(part 1 of 2)
# Autodesk Inventor assembly: #SHOOTER.3
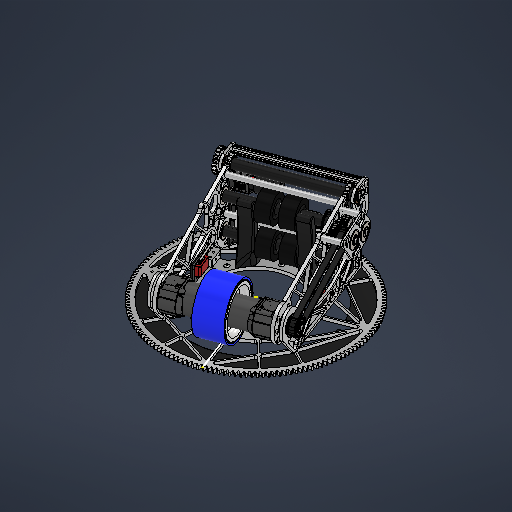
[picture p0: Inventor's stored thumbnail of the model, 512x512]
Saved by Autodesk Inventor 2026 (Build 300175000, 175)
## iProperties
Created: 2026-01-27
Part Number: #SHOOTER.3
Document SubType Name: Assembly
Designer: Owen L
Mass: 5085.84 g
Surface Area: 9899.41 cm^2
Volume: 1803.06 cm^3
Density: 2.82066 g/cm^3
Author: Owen L
## Documents named in this file (60)
- C:\Users\littl\OneDrive\Documents\GitHub\2026-Robot-Mechanical\Shooter\Shooter - Front Motors\#SHOOTER.FRONT_MOTORS.iam
- C:\Users\littl\OneDrive\Documents\GitHub\2026-Robot-Mechanical\Shooter\Shooter - Front Motors\PLATE,SHOOTER,SIDE.ipt
- C:\Users\littl\OneDrive\Documents\GitHub\2026-Robot-Mechanical\#1_CAD Library\Electronics\CONTROLS,SPARK_FLEX.ipt
- C:\Users\littl\OneDrive\Documents\GitHub\2026-Robot-Mechanical\#1_CAD Library\Power Transmission\Bushings\PURCHASED,BUSHING,13.75mmID,0.75inOD.ipt
- C:\Users\littl\OneDrive\Documents\GitHub\2026-Robot-Mechanical\#1_CAD Library\Power Transmission\Bearings\PURCHASED,HEX_BEARING.ipt
- C:\Users\littl\OneDrive\Documents\GitHub\2026-Robot-Mechanical\#1_CAD Library\Motors\MOTOR,REV,NEO,VORTEX.ipt
- C:\Users\littl\OneDrive\Documents\GitHub\2026-Robot-Mechanical\#1_CAD Library\Motors\MOTOR,REV,NEO,550.ipt
- C:\Users\littl\OneDrive\Documents\GitHub\2026-Robot-Mechanical\#1_CAD Library\Power Transmission\UltraPlanetary\PURCHASED,REV,ULTRAPLANETARY,2-STAGE.iam
- C:\Users\littl\OneDrive\Documents\GitHub\2026-Robot-Mechanical\Shooter\Shooter - Front Motors\#SHOOTER.3\Design Accelerator\PLATE,HOOD,SIDE.ipt
- C:\Users\littl\OneDrive\Documents\GitHub\2026-Robot-Mechanical\Shooter\Shooter - Front Motors\#SHOOTER.3\Design Accelerator\PLATE.HOOD,PINION,GEAR.ipt
- C:\Users\littl\OneDrive\Documents\GitHub\2026-Robot-Mechanical\Shooter\Shooter - Front Motors\STOCK,HEX,ROUND,HOOD.ipt
- C:\Users\littl\OneDrive\Documents\GitHub\2026-Robot-Mechanical\#1_CAD Library\Power Transmission\Pulleys\PURCHASED,HTD5mm,20T,PULLEY.ipt
- C:\Users\littl\OneDrive\Documents\GitHub\2026-Robot-Mechanical\Shooter\Shooter - Front Motors\#SHOOTER.3\Design Accelerator\PLATE,HOOD,DRIVE,GEAR,SHAFT.ipt
- C:\Users\littl\OneDrive\Documents\GitHub\2026-Robot-Mechanical\Shooter\Shooter - Front Motors\#SHOOTER.3\Design Accelerator\PLATE,HOOD,DRIVE,GEAR,MOTOR.ipt
- C:\Users\littl\OneDrive\Documents\GitHub\2026-Robot-Mechanical\Shooter\Shooter - Front Motors\STOCK,SHAFT,HEX,SHOOTER.ipt
- C:\Users\littl\OneDrive\Documents\GitHub\2026-Robot-Mechanical\Shooter\Shooter - Front Motors\PLATE,BEARING,MOUNT.ipt
- C:\Users\littl\OneDrive\Documents\GitHub\2026-Robot-Mechanical\Shooter\Shooter - Front Motors\STOCK,SHAFT,HEX,HOOD,WHEELS,LONG.ipt
- C:\Users\littl\OneDrive\Documents\GitHub\2026-Robot-Mechanical\Shooter\Shooter - Front Motors\STOCK,SHAFT,HEX,HOOD,REVERSER.ipt
- C:\Users\littl\OneDrive\Documents\GitHub\2026-Robot-Mechanical\Shooter\Shooter - Front Motors\STOCK,SHAFT,HEX,HOOD,WHEELS,SHORT.ipt
- C:\Users\littl\OneDrive\Documents\GitHub\2026-Robot-Mechanical\Shooter\Shooter - Front Motors\PLATE,SHOOTER,BOTTOM.ipt
- C:\Users\littl\OneDrive\Documents\GitHub\2026-Robot-Mechanical\Shooter\Shooter - Front Motors\PLATE,SHOOTER,BACK.ipt
- C:\Users\littl\OneDrive\Documents\GitHub\2026-Robot-Mechanical\Shooter\Shooter - Front Motors\STOCK,CHURRO,HEX,BACK.ipt
- C:\Users\littl\OneDrive\Documents\GitHub\2026-Robot-Mechanical\Shooter\Shooter - Front Motors\PURCHASED,WASHER.ipt
- C:\Users\littl\OneDrive\Documents\GitHub\2026-Robot-Mechanical\#1_CAD Library\Wheels\Shooter\PURCHASED,2inOD,HEX,SHOOTER,WHEEL.ipt
- C:\Users\littl\OneDrive\Documents\GitHub\2026-Robot-Mechanical\#1_CAD Library\Building Materials\Fasteners\Bolts\PURCHASED,0.25-20x0.5in,BUTTONHEAD,BOLT.ipt
- C:\Users\littl\OneDrive\Documents\GitHub\2026-Robot-Mechanical\#1_CAD Library\Building Materials\Fasteners\Bolts\PURCHASED,10-32x0.5in,BUTTONHEAD,BOLT.ipt
- C:\Users\littl\OneDrive\Documents\GitHub\2026-Robot-Mechanical\#1_CAD Library\Building Materials\Fasteners\Bolts\PURCHASED,M3x10mm,BUTTONHEAD,BOLT.ipt
- C:\Users\littl\OneDrive\Documents\GitHub\2026-Robot-Mechanical\Shooter\Shooter - Front Motors\3DPRINT,HOOD,DRIVEGEAR,SPACER.ipt
- C:\Users\littl\OneDrive\Documents\GitHub\2026-Robot-Mechanical\Shooter\Shooter - Front Motors\3DPRINT,REVERSERGEAR,SPACER.ipt
- C:\Users\littl\OneDrive\Documents\GitHub\2026-Robot-Mechanical\Shooter\Shooter - Front Motors\3DPRINT,BACKROLLERS,OPENSIDE,SPACER.ipt
- C:\Users\littl\OneDrive\Documents\GitHub\2026-Robot-Mechanical\Shooter\Shooter - Front Motors\3DPRINT,BACKROLLERS,PULLEYSIDE,SPACER.ipt
- C:\Users\littl\OneDrive\Documents\GitHub\2026-Robot-Mechanical\Shooter\Shooter - Front Motors\3DPRINT,BACKROLLERS,INTERROLLER,SPACER.ipt
- C:\Users\littl\OneDrive\Documents\GitHub\2026-Robot-Mechanical\#1_CAD Library\Power Transmission\Gears\PURCHASED,GEAR,20DP,30T,HEX.ipt
- C:\Users\littl\OneDrive\Documents\GitHub\2026-Robot-Mechanical\Shooter\Shooter - Front Motors\3DPRINT,BACKRAIL.ipt
- C:\Users\littl\OneDrive\Documents\GitHub\2026-Robot-Mechanical\Shooter\Shooter - Front Motors\3DPRINT,BACKRAIL_MIR.ipt
- C:\Users\littl\OneDrive\Documents\GitHub\2026-Robot-Mechanical\Shooter\Shooter - Front Motors\PLATE,NUTBLOCK.ipt
- C:\Users\littl\OneDrive\Documents\GitHub\2026-Robot-Mechanical\#1_CAD Library\Building Materials\Fasteners\Bolts\PURCHASED,M4x12mm,BUTTONHEAD,BOLT.ipt
- C:\Users\littl\OneDrive\Documents\GitHub\2026-Robot-Mechanical\Shooter\Shooter - Front Motors\STANDIN,45T,HTD5mm,BELT.ipt
- C:\Users\littl\OneDrive\Documents\GitHub\2026-Robot-Mechanical\Shooter\Shooter - Front Motors\STANDIN,90T,HTD5mm,BELT.ipt
- C:\Users\littl\OneDrive\Documents\GitHub\2026-Robot-Mechanical\Shooter\Shooter - Front Motors\3DPRINT,FLYWHEELTOHOOD,SPACER.ipt
- C:\Users\littl\OneDrive\Documents\GitHub\2026-Robot-Mechanical\Shooter\Shooter - Front Motors\STOCK,HOOD,SPACER,10-32,6.25in.ipt
- C:\Users\littl\OneDrive\Documents\GitHub\2026-Robot-Mechanical\Shooter\Shooter - Front Motors\3DPRINT,SIDEPLATETOHOOD,SPACER .ipt
- C:\Users\littl\OneDrive\Documents\GitHub\2026-Robot-Mechanical\Shooter\Shooter - Front Motors\3DPRINT,SIDEPLATETOHOODGEAR,SPACER.ipt
- C:\Users\littl\OneDrive\Documents\GitHub\2026-Robot-Mechanical\Shooter\Shooter - Front Motors\3DPRINT,BUSHINGTOHOODDRIVEGEAR,SPACER.ipt
- C:\Users\littl\OneDrive\Documents\GitHub\2026-Robot-Mechanical\Shooter\Shooter - Front Motors\3DPRINT,HOOD,ALIGNMENT,PLATES.ipt
- C:\Users\littl\OneDrive\Documents\GitHub\2026-Robot-Mechanical\#1_CAD Library\Building Materials\Fasteners\Bolts\PURCHASED,M3x16mm,BUTTONHEAD,BOLT.ipt
- C:\Users\littl\OneDrive\Documents\GitHub\2026-Robot-Mechanical\#1_CAD Library\Building Materials\Fasteners\Nuts\PURCHASED,M3,NYLOCK,NUT.ipt
- C:\Users\littl\OneDrive\Documents\GitHub\2026-Robot-Mechanical\#1_CAD Library\Electronics\CONTROLS,LIMIT_SWITCH,VEX.iam
- C:\Users\littl\OneDrive\Documents\GitHub\2026-Robot-Mechanical\Shooter\Shooter - Front Motors\3DPRINT,LIMIT_SWITCH,SPACER.ipt
- C:\Users\littl\OneDrive\Documents\GitHub\2026-Robot-Mechanical\Shooter\Shooter - Front Motors\3DPRINT,LIMIT_SWITCH,SPACER,RIGHT.ipt
- C:\Users\littl\OneDrive\Documents\GitHub\2026-Robot-Mechanical\Shooter\Shooter - Front Motors\PLATE,FLYWHEEL,HUB.ipt
- C:\Users\littl\OneDrive\Documents\GitHub\2026-Robot-Mechanical\Shooter\Shooter - Front Motors\CAST,FLYWHEEL,GRIP.ipt
- C:\Users\littl\OneDrive\Documents\GitHub\2026-Robot-Mechanical\#1_CAD Library\Electronics\CONTROLS,SPARK_MAX.ipt
- C:\Users\littl\OneDrive\Documents\GitHub\2026-Robot-Mechanical\Shooter\Shooter - Front Motors\3DPRINT,SPARK_MAX,MOUNT.ipt
- C:\Users\littl\OneDrive\Documents\GitHub\2026-Robot-Mechanical\#1_CAD Library\Building Materials\Fasteners\Bolts\PURCHASED,10-32x0.625in,FLATHEAD,BOLT.ipt
- C:\Users\littl\OneDrive\Documents\GitHub\2026-Robot-Mechanical\Shooter\Shooter - Front Motors\3DPRINT,REVERSERGEAR,SPACER,SHORT.ipt
- C:\Users\littl\OneDrive\Documents\GitHub\2026-Robot-Mechanical\Shooter\Shooter - Front Motors\3DPRINT,CABLE,GUARD.ipt
- C:\Users\littl\OneDrive\Documents\GitHub\2026-Robot-Mechanical\Shooter\Shooter - Front Motors\3DPRINT,BACKROLLERS,PULLEY,SPACER.ipt
- C:\Users\littl\OneDrive\Documents\GitHub\2026-Robot-Mechanical\Shooter\Shooter - Front Motors\PLATE,NUTBLOCK,BACK.ipt
- C:\Users\littl\OneDrive\Documents\GitHub\2026-Robot-Mechanical\Shooter\Shooter - Front Motors\STOCK,ROUND,0.375inOD,10-32,STANDOFF.ipt
## Components (209 placed, 59 different names)
1. STOCK,ROUND,0.375inOD,10-32,STANDOFF:1 — Insert:243
2. STOCK,ROUND,0.375inOD,10-32,STANDOFF:2 — Insert:244
3. STOCK,ROUND,0.375inOD,10-32,STANDOFF:3 — Insert:245
4. PLATE,NUTBLOCK,BACK:1 — Insert:238, Insert:239
5. PLATE,NUTBLOCK:1 — Insert:101, Insert:102
6. PLATE,NUTBLOCK:2 — Insert:103, Insert:104
7. PLATE,NUTBLOCK:4 — Insert:107, Mate:181
8. PLATE,NUTBLOCK:5 — Insert:110, Mate:193
9. STANDIN,45T,HTD5mm,BELT:1 — Mate:147, Mate:148, Mate:152
10. STANDIN,90T,HTD5mm,BELT:1 — Mate:149, Mate:150, Mate:151
11. CONTROLS,SPARK_FLEX:1 — Mate:3, Mate:4, Mate:5, Insert:188, Insert:219
12. CONTROLS,SPARK_FLEX:2 — Mate:12, Mate:13, Mate:14, Insert:191, Insert:220
13. MOTOR,REV,NEO,VORTEX:1 — Mate:3, Mate:4, Mate:5
14. MOTOR,REV,NEO,VORTEX:2 — Mate:12, Mate:13, Mate:14, Mate:209
15. MOTOR,REV,NEO,550:1 — Insert:1, Mate:1
16. CONTROLS,SPARK_MAX:1 — Mate:216, Mate:220, Mate:221
17. CONTROLS,LIMIT_SWITCH,VEX:2 [sub-assembly] — Mate:198, Mate:199, Mate:200, Mate:203, Mate:204
18. CONTROLS,LIMIT_SWITCH,VEX:1 [sub-assembly] — Mate:184, Mate:185, Mate:186, Mate:188, Mate:190
19. PURCHASED,BUSHING,13.75mmID,0.75inOD:1 — Insert:3, Mate:8, Mate:166, Mate:173
20. PURCHASED,BUSHING,13.75mmID,0.75inOD:2 — Insert:7, Mate:11, Mate:170
21. PURCHASED,HEX_BEARING:1 — Insert:4, Mate:30, Mate:31, Mate:191, Mate:192
22. PURCHASED,REV,ULTRAPLANETARY,2-STAGE:1 [sub-assembly] — Insert:1, Mate:1, Insert:2, Mate:2, Flush:1, Insert:14, Mate:26
23. PURCHASED,HTD5mm,20T,PULLEY:1 — Mate:59, Mate:60, Mate:97, Mate:152, Mate:248
24. PURCHASED,HEX_BEARING:5 — Insert:15, Mate:37, Mate:38, Flush:3, Mate:194
25. PURCHASED,HEX_BEARING:6 — Insert:16, Mate:39, Mate:40, Flush:4
26. PURCHASED,HEX_BEARING:7 — Insert:17, Mate:128
27. PURCHASED,HEX_BEARING:8 — Insert:18
28. PURCHASED,HEX_BEARING:9 — Insert:19, Mate:155
29. PURCHASED,HEX_BEARING:10 — Insert:20, Mate:162
30. PURCHASED,HEX_BEARING:11 — Insert:21, Mate:159
31. PURCHASED,HEX_BEARING:12 — Mate:41, Mate:42, Flush:5, Mate:129, Insert:231
32. PURCHASED,HEX_BEARING:14 — Mate:88, Mate:121, Mate:122, Insert:96
33. PURCHASED,HEX_BEARING:15 — Insert:94, Mate:226
34. PURCHASED,HTD5mm,20T,PULLEY:2 — Mate:61, Mate:62, Mate:100, Mate:246
35. PURCHASED,2inOD,HEX,SHOOTER,WHEEL:1 — Mate:65, Mate:66, Mate:73, Mate:103, Mate:243
36. PURCHASED,2inOD,HEX,SHOOTER,WHEEL:2 — Mate:67, Mate:68, Mate:73, Flush:8, Mate:91
37. PURCHASED,2inOD,HEX,SHOOTER,WHEEL:3 — Mate:69, Mate:70, Mate:74, Mate:106, Mate:244
38. PURCHASED,2inOD,HEX,SHOOTER,WHEEL:4 — Mate:71, Mate:72, Mate:74, Flush:8, Mate:94
39. PURCHASED,WASHER:12 — Insert:86, Insert:87
40. PURCHASED,GEAR,20DP,30T,HEX:1 — Mate:124, Mate:125, Mate:129, Mate:146
41. PURCHASED,GEAR,20DP,30T,HEX:2 — Mate:126, Mate:127, Mate:128
42. PURCHASED,HTD5mm,20T,PULLEY:3 — Mate:141, Mate:142, Flush:9
43. PURCHASED,HTD5mm,20T,PULLEY:4 — Mate:144, Mate:145, Mate:146, Mate:151, Mate:227
44. 3DPRINT,BACKROLLERS,PULLEY,SPACER:1 — Mate:245, Mate:246, Mate:250
45. 3DPRINT,BACKROLLERS,PULLEY,SPACER:2 — Mate:247, Mate:248, Mate:249
46. 3DPRINT,CABLE,GUARD:1 — Mate:228, Mate:229, Mate:230, Mate:237, Mate:238
47. 3DPRINT,CABLE,GUARD:2 — Mate:228, Mate:229, Mate:230, Mate:231, Mate:232, Mate:233
48. 3DPRINT,CABLE,GUARD:3 — Mate:231, Mate:232, Mate:233, Mate:234, Mate:235, Mate:236
49. 3DPRINT,CABLE,GUARD:4 — Mate:234, Mate:235, Mate:236, Mate:239
50. 3DPRINT,HOOD,DRIVEGEAR,SPACER:1 — Mate:83, Mate:84, Mate:85, Mate:163
51. 3DPRINT,REVERSERGEAR,SPACER:1 — Mate:86, Mate:87, Mate:88
52. 3DPRINT,BACKROLLERS,OPENSIDE,SPACER:1 — Mate:89, Mate:90, Mate:91, Mate:194
53. 3DPRINT,BACKROLLERS,OPENSIDE,SPACER:2 — Mate:92, Mate:93, Mate:94
54. 3DPRINT,BACKROLLERS,PULLEYSIDE,SPACER:1 — Mate:95, Mate:96, Mate:97, Mate:243
55. 3DPRINT,BACKROLLERS,PULLEYSIDE,SPACER:2 — Mate:98, Mate:99, Mate:100, Mate:244
56. 3DPRINT,BACKROLLERS,INTERROLLER,SPACER:1 — Mate:101, Mate:102, Mate:103
57. 3DPRINT,BACKROLLERS,INTERROLLER,SPACER:2 — Mate:104, Mate:105, Mate:106
58. 3DPRINT,BACKRAIL:1 — Mate:131, Mate:212, Mate:225
59. 3DPRINT,BACKRAIL_MIR:1 — Mate:240, Mate:241, Mate:242
60. 3DPRINT,FLYWHEELTOHOOD,SPACER:1 — Mate:153, Mate:154, Mate:155
61. 3DPRINT,SIDEPLATETOHOOD,SPACER :1 — Mate:157, Mate:158, Mate:159
62. 3DPRINT,SIDEPLATETOHOODGEAR,SPACER:1 — Mate:171, Mate:172, Mate:173
63. 3DPRINT,BUSHINGTOHOODDRIVEGEAR,SPACER:1 — Mate:164, Mate:165, Mate:166, Mate:167
64. 3DPRINT,SIDEPLATETOHOOD,SPACER :2 — Mate:160, Mate:161, Mate:162, Mate:192
65. 3DPRINT,BUSHINGTOHOODDRIVEGEAR,SPACER:2 — Mate:168, Mate:169, Mate:170
66. 3DPRINT,HOOD,ALIGNMENT,PLATES:1 — Insert:161, Insert:165, Insert:174, Insert:175, Insert:176, Insert:177, Insert:178
67. 3DPRINT,HOOD,ALIGNMENT,PLATES:2 — Insert:163, Insert:164, Insert:179, Insert:180, Insert:181, Insert:182, Insert:183
68. 3DPRINT,HOOD,ALIGNMENT,PLATES:3 — Insert:166, Insert:167, Insert:170, Insert:171, Insert:172, Insert:173
69. 3DPRINT,HOOD,ALIGNMENT,PLATES:4 — Insert:168, Insert:169, Insert:184, Insert:185, Insert:186, Insert:187
70. 3DPRINT,LIMIT_SWITCH,SPACER:1 — Mate:181, Mate:182, Mate:183, Mate:184, Mate:186, Flush:10
71. 3DPRINT,LIMIT_SWITCH,SPACER,RIGHT:1 — Mate:196, Mate:197, Mate:198, Mate:199, Mate:200, Flush:10
72. 3DPRINT,SPARK_MAX,MOUNT:1 — Mate:217, Mate:218, Mate:220, Mate:221, Mate:224, Insert:240, Insert:241, Insert:242
73. 3DPRINT,REVERSERGEAR,SPACER,SHORT:1 — Mate:226, Mate:227
74. PURCHASED,10-32x0.5in,BUTTONHEAD,BOLT:78 — Insert:240
75. PURCHASED,10-32x0.5in,BUTTONHEAD,BOLT:79 — Insert:241
76. PURCHASED,10-32x0.5in,BUTTONHEAD,BOLT:80 — Insert:242
77. PURCHASED,WASHER:2 — Insert:47, Insert:62
78. PURCHASED,WASHER:3 — Insert:48, Insert:64
79. PURCHASED,WASHER:4 — Insert:49, Insert:63
80. PURCHASED,WASHER:5 — Insert:50, Insert:65, Mate:191
81. PURCHASED,WASHER:6 — Insert:51, Insert:66
82. PURCHASED,WASHER:7 — Insert:52, Insert:67
83. PURCHASED,WASHER:8 — Insert:53, Insert:68
84. PURCHASED,WASHER:9 — Insert:54, Insert:69
85. PURCHASED,WASHER:10 — Insert:55, Insert:70
86. PURCHASED,M3,NYLOCK,NUT:3 — Insert:187
87. PURCHASED,M3,NYLOCK,NUT:5 — Insert:185
88. PURCHASED,M3,NYLOCK,NUT:6 — Insert:184
89. PURCHASED,M3,NYLOCK,NUT:7 — Insert:183
90. PURCHASED,M3,NYLOCK,NUT:1 — Insert:186
91. PURCHASED,M3,NYLOCK,NUT:8 — Insert:182
92. PURCHASED,M3,NYLOCK,NUT:9 — Insert:181
93. PURCHASED,M3,NYLOCK,NUT:10 — Insert:180
94. PURCHASED,M3,NYLOCK,NUT:11 — Insert:179
95. PURCHASED,0.25-20x0.5in,BUTTONHEAD,BOLT:1 — Insert:146
96. PURCHASED,0.25-20x0.5in,BUTTONHEAD,BOLT:4 — Insert:145
97. PURCHASED,M3x10mm,BUTTONHEAD,BOLT:1 — Insert:77
98. PURCHASED,10-32x0.5in,BUTTONHEAD,BOLT:6 — Insert:62
99. PURCHASED,10-32x0.5in,BUTTONHEAD,BOLT:7 — Insert:63
100. PURCHASED,10-32x0.5in,BUTTONHEAD,BOLT:8 — Insert:65
101. PURCHASED,10-32x0.5in,BUTTONHEAD,BOLT:9 — Insert:64
102. PURCHASED,10-32x0.5in,BUTTONHEAD,BOLT:10 — Insert:66
103. PURCHASED,10-32x0.5in,BUTTONHEAD,BOLT:11 — Insert:67
104. PURCHASED,10-32x0.5in,BUTTONHEAD,BOLT:12 — Insert:68
105. PURCHASED,10-32x0.5in,BUTTONHEAD,BOLT:13 — Insert:69
106. PURCHASED,10-32x0.5in,BUTTONHEAD,BOLT:14 — Insert:70
107. PURCHASED,10-32x0.5in,BUTTONHEAD,BOLT:16 — Insert:87
108. PURCHASED,M3x10mm,BUTTONHEAD,BOLT:2 — Insert:78
109. PURCHASED,M3x10mm,BUTTONHEAD,BOLT:3 — Insert:80
110. PURCHASED,M3x10mm,BUTTONHEAD,BOLT:4 — Insert:79
111. PURCHASED,M3x10mm,BUTTONHEAD,BOLT:5 — Insert:81
112. PURCHASED,M3x10mm,BUTTONHEAD,BOLT:6 — Insert:82
113. PURCHASED,M3x10mm,BUTTONHEAD,BOLT:7 — Insert:83
114. PURCHASED,M3x10mm,BUTTONHEAD,BOLT:8 — Insert:84
115. PURCHASED,M3x10mm,BUTTONHEAD,BOLT:9 — Insert:85
116. PURCHASED,10-32x0.5in,BUTTONHEAD,BOLT:21 — Insert:99
117. PURCHASED,10-32x0.5in,BUTTONHEAD,BOLT:22 — Insert:98
118. PURCHASED,10-32x0.5in,BUTTONHEAD,BOLT:23 — Insert:100
119. PURCHASED,10-32x0.5in,BUTTONHEAD,BOLT:24 — Insert:91
120. PURCHASED,10-32x0.5in,BUTTONHEAD,BOLT:25 — Insert:92
121. PURCHASED,10-32x0.5in,BUTTONHEAD,BOLT:26 — Insert:93
122. PURCHASED,10-32x0.5in,BUTTONHEAD,BOLT:27 — Insert:114
123. PURCHASED,10-32x0.5in,BUTTONHEAD,BOLT:28 — Insert:113
124. PURCHASED,10-32x0.5in,BUTTONHEAD,BOLT:29 — Insert:112
125. PURCHASED,10-32x0.5in,BUTTONHEAD,BOLT:30 — Insert:111
126. PURCHASED,10-32x0.5in,BUTTONHEAD,BOLT:31 — Insert:115
127. PURCHASED,10-32x0.5in,BUTTONHEAD,BOLT:32 — Insert:116
128. PURCHASED,10-32x0.5in,BUTTONHEAD,BOLT:33 — Insert:117
129. PURCHASED,10-32x0.5in,BUTTONHEAD,BOLT:34 — Insert:118
130. PURCHASED,10-32x0.5in,BUTTONHEAD,BOLT:35 — Insert:119
131. PURCHASED,10-32x0.5in,BUTTONHEAD,BOLT:36 — Insert:120
132. PURCHASED,10-32x0.5in,BUTTONHEAD,BOLT:37 — Insert:121
133. PURCHASED,10-32x0.5in,BUTTONHEAD,BOLT:38 — Insert:122
134. PURCHASED,10-32x0.5in,BUTTONHEAD,BOLT:40 — Insert:124
135. PURCHASED,10-32x0.5in,BUTTONHEAD,BOLT:41 — Insert:125
136. PURCHASED,10-32x0.5in,BUTTONHEAD,BOLT:42 — Insert:126
137. PURCHASED,10-32x0.5in,BUTTONHEAD,BOLT:43 — Insert:127
138. PURCHASED,10-32x0.5in,BUTTONHEAD,BOLT:44 — Insert:128
139. PURCHASED,10-32x0.5in,BUTTONHEAD,BOLT:45 — Insert:129
140. PURCHASED,M4x12mm,BUTTONHEAD,BOLT:1 — Insert:137, Insert:232
141. PURCHASED,M4x12mm,BUTTONHEAD,BOLT:2 — Insert:138, Mate:212
142. PURCHASED,M4x12mm,BUTTONHEAD,BOLT:3 — Insert:139, Insert:234
143. PURCHASED,M4x12mm,BUTTONHEAD,BOLT:4 — Insert:140, Insert:233
144. PURCHASED,M4x12mm,BUTTONHEAD,BOLT:5 — Insert:141, Insert:237
145. PURCHASED,M4x12mm,BUTTONHEAD,BOLT:6 — Insert:142
146. PURCHASED,M4x12mm,BUTTONHEAD,BOLT:7 — Insert:143, Insert:236
147. PURCHASED,M4x12mm,BUTTONHEAD,BOLT:8 — Insert:144, Insert:235
148. PURCHASED,10-32x0.5in,BUTTONHEAD,BOLT:49 — Insert:154
149. PURCHASED,10-32x0.5in,BUTTONHEAD,BOLT:50 — Insert:156
150. PURCHASED,10-32x0.5in,BUTTONHEAD,BOLT:51 — Insert:155
151. PURCHASED,10-32x0.5in,BUTTONHEAD,BOLT:52 — Insert:157
152. PURCHASED,M3x16mm,BUTTONHEAD,BOLT:1 — Insert:170
153. PURCHASED,M3x16mm,BUTTONHEAD,BOLT:2 — Insert:171
154. PURCHASED,M3x16mm,BUTTONHEAD,BOLT:3 — Insert:172
155. PURCHASED,M3x16mm,BUTTONHEAD,BOLT:4 — Insert:173
156. PURCHASED,M3x16mm,BUTTONHEAD,BOLT:5 — Insert:174
157. PURCHASED,M3x16mm,BUTTONHEAD,BOLT:6 — Insert:175
158. PURCHASED,M3x16mm,BUTTONHEAD,BOLT:7 — Insert:176
159. PURCHASED,M3x16mm,BUTTONHEAD,BOLT:8 — Insert:177
160. PURCHASED,M3x16mm,BUTTONHEAD,BOLT:9 — Insert:178
161. PURCHASED,M4x12mm,BUTTONHEAD,BOLT:9 — Mate:187, Mate:188
162. PURCHASED,M4x12mm,BUTTONHEAD,BOLT:10 — Mate:189, Mate:190
163. PURCHASED,10-32x0.5in,BUTTONHEAD,BOLT:53 — Insert:195
164. PURCHASED,10-32x0.5in,BUTTONHEAD,BOLT:56 — Insert:198
165. PURCHASED,10-32x0.5in,BUTTONHEAD,BOLT:57 — Insert:201
166. PURCHASED,10-32x0.5in,BUTTONHEAD,BOLT:58 — Insert:200
167. PURCHASED,10-32x0.5in,BUTTONHEAD,BOLT:59 — Insert:199
168. PURCHASED,10-32x0.5in,BUTTONHEAD,BOLT:60 — Insert:203
169. PURCHASED,10-32x0.5in,BUTTONHEAD,BOLT:61 — Insert:204
170. PURCHASED,10-32x0.5in,BUTTONHEAD,BOLT:62 — Insert:202
171. PURCHASED,10-32x0.5in,BUTTONHEAD,BOLT:63 — Insert:205
172. PURCHASED,10-32x0.5in,BUTTONHEAD,BOLT:64 — Insert:207
173. PURCHASED,10-32x0.5in,BUTTONHEAD,BOLT:65 — Insert:208
174. PURCHASED,10-32x0.5in,BUTTONHEAD,BOLT:66 — Insert:206
175. PURCHASED,10-32x0.5in,BUTTONHEAD,BOLT:67 — Insert:210
176. PURCHASED,10-32x0.5in,BUTTONHEAD,BOLT:68 — Insert:209
177. PURCHASED,M4x12mm,BUTTONHEAD,BOLT:11 — Mate:201, Mate:204
178. PURCHASED,M4x12mm,BUTTONHEAD,BOLT:12 — Mate:202, Mate:203
179. PURCHASED,10-32x0.625in,FLATHEAD,BOLT:1 — Insert:221
180. PURCHASED,10-32x0.5in,BUTTONHEAD,BOLT:69 — Insert:222
181. PURCHASED,10-32x0.5in,BUTTONHEAD,BOLT:70 — Insert:223
182. PURCHASED,10-32x0.5in,BUTTONHEAD,BOLT:71 — Insert:224
183. PURCHASED,10-32x0.5in,BUTTONHEAD,BOLT:72 — Insert:225
184. PURCHASED,10-32x0.5in,BUTTONHEAD,BOLT:73 — Insert:226
185. PURCHASED,10-32x0.5in,BUTTONHEAD,BOLT:74 — Insert:227
186. PURCHASED,10-32x0.5in,BUTTONHEAD,BOLT:75 — Insert:228
187. PURCHASED,10-32x0.5in,BUTTONHEAD,BOLT:76 — Insert:229
188. PURCHASED,10-32x0.5in,BUTTONHEAD,BOLT:77 — Insert:230
189. PLATE,FLYWHEEL,HUB:1 — Mate:207, Mate:208, Mate:209, Mate:214, Flush:12, Mate:215
190. PLATE,HOOD,SIDE:1 — Mate:6, Mate:7, Mate:15, Insert:15, Insert:16, Mate:27, Insert:20, Insert:152, Insert:154, Insert:155, Mate:174, Insert:161, Insert:163, Insert:164, Insert:165, Insert:188, Insert:205, Insert:206, Insert:207, Insert:208, Insert:209, Insert:210, Insert:219
191. PLATE.HOOD,PINION,GEAR:1 — Mate:22, Mate:23, Mate:163, Mate:167
192. PLATE,HOOD,SIDE:2 — Mate:7, Mate:15, Insert:17, Insert:18, Mate:27, Insert:21, Insert:91, Insert:92, Insert:93, Mate:147, Mate:148, Mate:150, Insert:153, Insert:156, Insert:157, Insert:166, Insert:167, Insert:168, Insert:169, Insert:191, Insert:199, Insert:200, Insert:201, Insert:202, Insert:203, Insert:204, Insert:220, Insert:231, Insert:243, Insert:244, Insert:245
193. PLATE.HOOD,PINION,GEAR:2 — Mate:20, Mate:21, Mate:85
194. PLATE,HOOD,DRIVE,GEAR,SHAFT:1 — Mate:24, Mate:25, Flush:2
195. PLATE,HOOD,DRIVE,GEAR,MOTOR:1 — Insert:14, Mate:26, Flush:2, Insert:77, Insert:78, Insert:79, Insert:80, Insert:81
196. PLATE,SHOOTER,SIDE:1 — Insert:2, Mate:2, Insert:3, Insert:4, Mate:6, Mate:36, Insert:82, Insert:83, Insert:84, Insert:85, Mate:120, Insert:110, Insert:111, Insert:112, Insert:113, Insert:114, Insert:146, Mate:182, Mate:187, Mate:189, Insert:195, Insert:229
197. PLATE,SHOOTER,BACK:1 — Insert:128, Insert:129, Insert:192, Insert:193, Mate:216, Mate:217, Mate:218, Mate:224, Insert:238, Insert:239
198. PLATE,SHOOTER,BOTTOM:1 — Mate:120, Mate:131, Insert:102, Insert:103, Insert:107, Insert:115, Insert:116, Insert:117, Insert:118, Insert:119, Insert:120, Insert:121, Insert:122, Insert:137, Insert:138, Insert:139, Insert:140, Insert:141, Insert:142, Insert:143, Insert:144, Mate:174, Mate:183, Mate:185, Mate:193, Mate:210, Mate:211, Mate:225, Insert:221, Insert:222, Insert:223, Insert:224, Insert:225, Insert:226, Insert:227, Insert:228, Mate:237, Mate:238, Mate:239, Insert:232, Insert:233, Insert:234, Insert:235, Insert:236, Insert:237, Mate:240, Mate:241, Mate:242
199. PLATE,BEARING,MOUNT:1 — Insert:94, Insert:96, Insert:98, Insert:99, Insert:100
200. PLATE,SHOOTER,SIDE:2 — Insert:7, Insert:19, Mate:36, Insert:40, Insert:101, Insert:104, Insert:124, Insert:125, Insert:126, Insert:127, Insert:145, Mate:149, Insert:192, Insert:193, Insert:198, Mate:196, Mate:197, Mate:201, Mate:202, Insert:230
201. STOCK,HEX,ROUND,HOOD:1 — Mate:8, Flush:1, Mate:11, Mate:20, Mate:21, Mate:22, Mate:23, Mate:24, Mate:25, Insert:47, Insert:55, Mate:83, Mate:84, Mate:164, Mate:165, Mate:168, Mate:169, Mate:171, Mate:172
202. STOCK,SHAFT,HEX,SHOOTER:1 — Mate:30, Mate:31, Insert:50, Insert:51, Mate:141, Mate:142, Flush:9, Mate:153, Mate:154, Mate:157, Mate:158, Mate:160, Mate:161, Mate:207, Mate:208, Rotation:4
203. STOCK,SHAFT,HEX,HOOD,WHEELS,LONG:1 — Mate:37, Mate:38, Flush:3, Mate:59, Mate:60, Insert:48, Insert:53, Mate:65, Mate:66, Mate:67, Mate:68, Mate:86, Mate:87, Mate:89, Mate:90, Mate:95, Mate:96, Mate:101, Mate:102, Mate:121, Mate:122, Mate:126, Mate:127, Rotation:1, Rotation:2, Rotation:3, Mate:247, Mate:249
204. STOCK,SHAFT,HEX,HOOD,REVERSER:1 — Mate:41, Mate:42, Flush:5, Insert:52, Insert:86, Mate:124, Mate:125, Mate:144, Mate:145, Rotation:1, Rotation:2, Rotation:4
205. STOCK,SHAFT,HEX,HOOD,WHEELS,SHORT:1 — Mate:39, Mate:40, Flush:4, Mate:61, Mate:62, Insert:49, Insert:54, Mate:69, Mate:70, Mate:71, Mate:72, Mate:92, Mate:93, Mate:98, Mate:99, Mate:104, Mate:105, Rotation:3, Mate:245, Mate:250
206. STOCK,CHURRO,HEX,BACK:1 — Insert:40
207. STOCK,HOOD,SPACER,10-32,6.25in:1 — Insert:152
208. STOCK,HOOD,SPACER,10-32,6.25in:2 — Insert:153
209. CAST,FLYWHEEL,GRIP:2 — Mate:214, Flush:12, Mate:215
## Relationships (348: Mate 173, Insert 162, Flush 9, RelateRotation 4)
- Insert:1: MOTOR,REV,NEO,550:1 ↔ PURCHASED,REV,ULTRAPLANETARY,2-STAGE:1
- Mate:1: MOTOR,REV,NEO,550:1 ↔ PURCHASED,REV,ULTRAPLANETARY,2-STAGE:1
- Insert:2: PURCHASED,REV,ULTRAPLANETARY,2-STAGE:1 ↔ PLATE,SHOOTER,SIDE:1
- Mate:2: PURCHASED,REV,ULTRAPLANETARY,2-STAGE:1 ↔ PLATE,SHOOTER,SIDE:1
- Insert:3: PURCHASED,BUSHING,13.75mmID,0.75inOD:1 ↔ PLATE,SHOOTER,SIDE:1
- Insert:4: PURCHASED,HEX_BEARING:1 ↔ PLATE,SHOOTER,SIDE:1
- Mate:3: CONTROLS,SPARK_FLEX:1 ↔ MOTOR,REV,NEO,VORTEX:1
- Mate:4: CONTROLS,SPARK_FLEX:1 ↔ MOTOR,REV,NEO,VORTEX:1
- Mate:5: CONTROLS,SPARK_FLEX:1 ↔ MOTOR,REV,NEO,VORTEX:1
- Mate:6: PLATE,HOOD,SIDE:1 ↔ PLATE,SHOOTER,SIDE:1
- Mate:7 (177.8 mm): PLATE,HOOD,SIDE:1 ↔ PLATE,HOOD,SIDE:2
- Mate:8: PURCHASED,BUSHING,13.75mmID,0.75inOD:1 ↔ STOCK,HEX,ROUND,HOOD:1
- Flush:1 (-6.35 mm): PURCHASED,REV,ULTRAPLANETARY,2-STAGE:1 ↔ STOCK,HEX,ROUND,HOOD:1
- Insert:7: PURCHASED,BUSHING,13.75mmID,0.75inOD:2 ↔ PLATE,SHOOTER,SIDE:2
- Mate:11: PURCHASED,BUSHING,13.75mmID,0.75inOD:2 ↔ STOCK,HEX,ROUND,HOOD:1
- Mate:12: CONTROLS,SPARK_FLEX:2 ↔ MOTOR,REV,NEO,VORTEX:2
- Mate:13: CONTROLS,SPARK_FLEX:2 ↔ MOTOR,REV,NEO,VORTEX:2
- Mate:14: CONTROLS,SPARK_FLEX:2 ↔ MOTOR,REV,NEO,VORTEX:2
- Mate:15: PLATE,HOOD,SIDE:1 ↔ PLATE,HOOD,SIDE:2
- Mate:20: PLATE.HOOD,PINION,GEAR:2 ↔ STOCK,HEX,ROUND,HOOD:1
- Mate:21: PLATE.HOOD,PINION,GEAR:2 ↔ STOCK,HEX,ROUND,HOOD:1
- Mate:22: PLATE.HOOD,PINION,GEAR:1 ↔ STOCK,HEX,ROUND,HOOD:1
- Mate:23: PLATE.HOOD,PINION,GEAR:1 ↔ STOCK,HEX,ROUND,HOOD:1
- Mate:24: PLATE,HOOD,DRIVE,GEAR,SHAFT:1 ↔ STOCK,HEX,ROUND,HOOD:1
- Mate:25: PLATE,HOOD,DRIVE,GEAR,SHAFT:1 ↔ STOCK,HEX,ROUND,HOOD:1
- Insert:14: PURCHASED,REV,ULTRAPLANETARY,2-STAGE:1 ↔ PLATE,HOOD,DRIVE,GEAR,MOTOR:1
- Mate:26: PURCHASED,REV,ULTRAPLANETARY,2-STAGE:1 ↔ PLATE,HOOD,DRIVE,GEAR,MOTOR:1
- Flush:2: PLATE,HOOD,DRIVE,GEAR,SHAFT:1 ↔ PLATE,HOOD,DRIVE,GEAR,MOTOR:1
- Insert:15: PURCHASED,HEX_BEARING:5 ↔ PLATE,HOOD,SIDE:1
- Insert:16: PURCHASED,HEX_BEARING:6 ↔ PLATE,HOOD,SIDE:1
- Insert:17: PURCHASED,HEX_BEARING:7 ↔ PLATE,HOOD,SIDE:2
- Insert:18: PURCHASED,HEX_BEARING:8 ↔ PLATE,HOOD,SIDE:2
- Mate:27: PLATE,HOOD,SIDE:1 ↔ PLATE,HOOD,SIDE:2
- Mate:30: PURCHASED,HEX_BEARING:1 ↔ STOCK,SHAFT,HEX,SHOOTER:1
- Mate:31: PURCHASED,HEX_BEARING:1 ↔ STOCK,SHAFT,HEX,SHOOTER:1
- Insert:19: PURCHASED,HEX_BEARING:9 ↔ PLATE,SHOOTER,SIDE:2
- Insert:20: PURCHASED,HEX_BEARING:10 ↔ PLATE,HOOD,SIDE:1
- Insert:21: PURCHASED,HEX_BEARING:11 ↔ PLATE,HOOD,SIDE:2
- Mate:36: PLATE,SHOOTER,SIDE:1 ↔ PLATE,SHOOTER,SIDE:2
- Mate:37: PURCHASED,HEX_BEARING:5 ↔ STOCK,SHAFT,HEX,HOOD,WHEELS,LONG:1
- Mate:38: PURCHASED,HEX_BEARING:5 ↔ STOCK,SHAFT,HEX,HOOD,WHEELS,LONG:1
- Flush:3: PURCHASED,HEX_BEARING:5 ↔ STOCK,SHAFT,HEX,HOOD,WHEELS,LONG:1
- Mate:39: PURCHASED,HEX_BEARING:6 ↔ STOCK,SHAFT,HEX,HOOD,WHEELS,SHORT:1
- Mate:40: PURCHASED,HEX_BEARING:6 ↔ STOCK,SHAFT,HEX,HOOD,WHEELS,SHORT:1
- Flush:4: PURCHASED,HEX_BEARING:6 ↔ STOCK,SHAFT,HEX,HOOD,WHEELS,SHORT:1
- Mate:41: PURCHASED,HEX_BEARING:12 ↔ STOCK,SHAFT,HEX,HOOD,REVERSER:1
- Mate:42: PURCHASED,HEX_BEARING:12 ↔ STOCK,SHAFT,HEX,HOOD,REVERSER:1
- Flush:5: PURCHASED,HEX_BEARING:12 ↔ STOCK,SHAFT,HEX,HOOD,REVERSER:1
- Mate:59: PURCHASED,HTD5mm,20T,PULLEY:1 ↔ STOCK,SHAFT,HEX,HOOD,WHEELS,LONG:1
- Mate:60: PURCHASED,HTD5mm,20T,PULLEY:1 ↔ STOCK,SHAFT,HEX,HOOD,WHEELS,LONG:1
- Mate:61: PURCHASED,HTD5mm,20T,PULLEY:2 ↔ STOCK,SHAFT,HEX,HOOD,WHEELS,SHORT:1
- Mate:62: PURCHASED,HTD5mm,20T,PULLEY:2 ↔ STOCK,SHAFT,HEX,HOOD,WHEELS,SHORT:1
- Insert:40: PLATE,SHOOTER,SIDE:2 ↔ STOCK,CHURRO,HEX,BACK:1
- Insert:47: PURCHASED,WASHER:2 ↔ STOCK,HEX,ROUND,HOOD:1
- Insert:48: PURCHASED,WASHER:3 ↔ STOCK,SHAFT,HEX,HOOD,WHEELS,LONG:1
- Insert:49: PURCHASED,WASHER:4 ↔ STOCK,SHAFT,HEX,HOOD,WHEELS,SHORT:1
- Insert:50: PURCHASED,WASHER:5 ↔ STOCK,SHAFT,HEX,SHOOTER:1
- Insert:51: PURCHASED,WASHER:6 ↔ STOCK,SHAFT,HEX,SHOOTER:1
- Insert:52: PURCHASED,WASHER:7 ↔ STOCK,SHAFT,HEX,HOOD,REVERSER:1
- Insert:53: PURCHASED,WASHER:8 ↔ STOCK,SHAFT,HEX,HOOD,WHEELS,LONG:1
- Insert:54: PURCHASED,WASHER:9 ↔ STOCK,SHAFT,HEX,HOOD,WHEELS,SHORT:1
- Insert:55: PURCHASED,WASHER:10 ↔ STOCK,HEX,ROUND,HOOD:1
- Mate:65: PURCHASED,2inOD,HEX,SHOOTER,WHEEL:1 ↔ STOCK,SHAFT,HEX,HOOD,WHEELS,LONG:1
- Mate:66: PURCHASED,2inOD,HEX,SHOOTER,WHEEL:1 ↔ STOCK,SHAFT,HEX,HOOD,WHEELS,LONG:1
- Mate:67: PURCHASED,2inOD,HEX,SHOOTER,WHEEL:2 ↔ STOCK,SHAFT,HEX,HOOD,WHEELS,LONG:1
- Mate:68: PURCHASED,2inOD,HEX,SHOOTER,WHEEL:2 ↔ STOCK,SHAFT,HEX,HOOD,WHEELS,LONG:1
- Mate:69: PURCHASED,2inOD,HEX,SHOOTER,WHEEL:3 ↔ STOCK,SHAFT,HEX,HOOD,WHEELS,SHORT:1
- Mate:70: PURCHASED,2inOD,HEX,SHOOTER,WHEEL:3 ↔ STOCK,SHAFT,HEX,HOOD,WHEELS,SHORT:1
- Mate:71: PURCHASED,2inOD,HEX,SHOOTER,WHEEL:4 ↔ STOCK,SHAFT,HEX,HOOD,WHEELS,SHORT:1
- Mate:72: PURCHASED,2inOD,HEX,SHOOTER,WHEEL:4 ↔ STOCK,SHAFT,HEX,HOOD,WHEELS,SHORT:1
- Mate:73 (12.7 mm): PURCHASED,2inOD,HEX,SHOOTER,WHEEL:1 ↔ PURCHASED,2inOD,HEX,SHOOTER,WHEEL:2
- Mate:74 (12.7 mm): PURCHASED,2inOD,HEX,SHOOTER,WHEEL:3 ↔ PURCHASED,2inOD,HEX,SHOOTER,WHEEL:4
- Insert:62: PURCHASED,WASHER:2 ↔ PURCHASED,10-32x0.5in,BUTTONHEAD,BOLT:6
- Insert:63: PURCHASED,WASHER:4 ↔ PURCHASED,10-32x0.5in,BUTTONHEAD,BOLT:7
- Insert:64: PURCHASED,WASHER:3 ↔ PURCHASED,10-32x0.5in,BUTTONHEAD,BOLT:9
- Insert:65: PURCHASED,WASHER:5 ↔ PURCHASED,10-32x0.5in,BUTTONHEAD,BOLT:8
- Insert:66: PURCHASED,WASHER:6 ↔ PURCHASED,10-32x0.5in,BUTTONHEAD,BOLT:10
- Insert:67: PURCHASED,WASHER:7 ↔ PURCHASED,10-32x0.5in,BUTTONHEAD,BOLT:11
- Insert:68: PURCHASED,WASHER:8 ↔ PURCHASED,10-32x0.5in,BUTTONHEAD,BOLT:12
- Insert:69: PURCHASED,WASHER:9 ↔ PURCHASED,10-32x0.5in,BUTTONHEAD,BOLT:13
- Insert:70: PURCHASED,WASHER:10 ↔ PURCHASED,10-32x0.5in,BUTTONHEAD,BOLT:14
- Insert:77: PURCHASED,M3x10mm,BUTTONHEAD,BOLT:1 ↔ PLATE,HOOD,DRIVE,GEAR,MOTOR:1
- Insert:78: PURCHASED,M3x10mm,BUTTONHEAD,BOLT:2 ↔ PLATE,HOOD,DRIVE,GEAR,MOTOR:1
- Insert:79: PURCHASED,M3x10mm,BUTTONHEAD,BOLT:4 ↔ PLATE,HOOD,DRIVE,GEAR,MOTOR:1
- Insert:80: PURCHASED,M3x10mm,BUTTONHEAD,BOLT:3 ↔ PLATE,HOOD,DRIVE,GEAR,MOTOR:1
- Insert:81: PURCHASED,M3x10mm,BUTTONHEAD,BOLT:5 ↔ PLATE,HOOD,DRIVE,GEAR,MOTOR:1
- Insert:82: PURCHASED,M3x10mm,BUTTONHEAD,BOLT:6 ↔ PLATE,SHOOTER,SIDE:1
- Insert:83: PURCHASED,M3x10mm,BUTTONHEAD,BOLT:7 ↔ PLATE,SHOOTER,SIDE:1
- Insert:84: PURCHASED,M3x10mm,BUTTONHEAD,BOLT:8 ↔ PLATE,SHOOTER,SIDE:1
- Insert:85: PURCHASED,M3x10mm,BUTTONHEAD,BOLT:9 ↔ PLATE,SHOOTER,SIDE:1
- Flush:8: PURCHASED,2inOD,HEX,SHOOTER,WHEEL:2 ↔ PURCHASED,2inOD,HEX,SHOOTER,WHEEL:4
- Mate:83: 3DPRINT,HOOD,DRIVEGEAR,SPACER:1 ↔ STOCK,HEX,ROUND,HOOD:1
- Mate:84: 3DPRINT,HOOD,DRIVEGEAR,SPACER:1 ↔ STOCK,HEX,ROUND,HOOD:1
- Mate:85: 3DPRINT,HOOD,DRIVEGEAR,SPACER:1 ↔ PLATE.HOOD,PINION,GEAR:2
- Mate:86: 3DPRINT,REVERSERGEAR,SPACER:1 ↔ STOCK,SHAFT,HEX,HOOD,WHEELS,LONG:1
- Mate:87: 3DPRINT,REVERSERGEAR,SPACER:1 ↔ STOCK,SHAFT,HEX,HOOD,WHEELS,LONG:1
- Mate:88: PURCHASED,HEX_BEARING:14 ↔ 3DPRINT,REVERSERGEAR,SPACER:1
- Mate:89: 3DPRINT,BACKROLLERS,OPENSIDE,SPACER:1 ↔ STOCK,SHAFT,HEX,HOOD,WHEELS,LONG:1
- Mate:90: 3DPRINT,BACKROLLERS,OPENSIDE,SPACER:1 ↔ STOCK,SHAFT,HEX,HOOD,WHEELS,LONG:1
- Mate:91: PURCHASED,2inOD,HEX,SHOOTER,WHEEL:2 ↔ 3DPRINT,BACKROLLERS,OPENSIDE,SPACER:1
- Mate:92: 3DPRINT,BACKROLLERS,OPENSIDE,SPACER:2 ↔ STOCK,SHAFT,HEX,HOOD,WHEELS,SHORT:1
- Mate:93: 3DPRINT,BACKROLLERS,OPENSIDE,SPACER:2 ↔ STOCK,SHAFT,HEX,HOOD,WHEELS,SHORT:1
- Mate:94: PURCHASED,2inOD,HEX,SHOOTER,WHEEL:4 ↔ 3DPRINT,BACKROLLERS,OPENSIDE,SPACER:2
- Mate:95: 3DPRINT,BACKROLLERS,PULLEYSIDE,SPACER:1 ↔ STOCK,SHAFT,HEX,HOOD,WHEELS,LONG:1
- Mate:96: 3DPRINT,BACKROLLERS,PULLEYSIDE,SPACER:1 ↔ STOCK,SHAFT,HEX,HOOD,WHEELS,LONG:1
- Mate:97: PURCHASED,HTD5mm,20T,PULLEY:1 ↔ 3DPRINT,BACKROLLERS,PULLEYSIDE,SPACER:1
- Mate:98: 3DPRINT,BACKROLLERS,PULLEYSIDE,SPACER:2 ↔ STOCK,SHAFT,HEX,HOOD,WHEELS,SHORT:1
- Mate:99: 3DPRINT,BACKROLLERS,PULLEYSIDE,SPACER:2 ↔ STOCK,SHAFT,HEX,HOOD,WHEELS,SHORT:1
- Mate:100: PURCHASED,HTD5mm,20T,PULLEY:2 ↔ 3DPRINT,BACKROLLERS,PULLEYSIDE,SPACER:2
- Mate:101: 3DPRINT,BACKROLLERS,INTERROLLER,SPACER:1 ↔ STOCK,SHAFT,HEX,HOOD,WHEELS,LONG:1
- Mate:102: 3DPRINT,BACKROLLERS,INTERROLLER,SPACER:1 ↔ STOCK,SHAFT,HEX,HOOD,WHEELS,LONG:1
- Mate:103: PURCHASED,2inOD,HEX,SHOOTER,WHEEL:1 ↔ 3DPRINT,BACKROLLERS,INTERROLLER,SPACER:1
- Mate:104: 3DPRINT,BACKROLLERS,INTERROLLER,SPACER:2 ↔ STOCK,SHAFT,HEX,HOOD,WHEELS,SHORT:1
- Mate:105: 3DPRINT,BACKROLLERS,INTERROLLER,SPACER:2 ↔ STOCK,SHAFT,HEX,HOOD,WHEELS,SHORT:1
- Mate:106: PURCHASED,2inOD,HEX,SHOOTER,WHEEL:3 ↔ 3DPRINT,BACKROLLERS,INTERROLLER,SPACER:2
- Insert:86: PURCHASED,WASHER:12 ↔ STOCK,SHAFT,HEX,HOOD,REVERSER:1
- Insert:87: PURCHASED,WASHER:12 ↔ PURCHASED,10-32x0.5in,BUTTONHEAD,BOLT:16
- Insert:91: PURCHASED,10-32x0.5in,BUTTONHEAD,BOLT:24 ↔ PLATE,HOOD,SIDE:2
- Insert:92: PURCHASED,10-32x0.5in,BUTTONHEAD,BOLT:25 ↔ PLATE,HOOD,SIDE:2
- Insert:93: PURCHASED,10-32x0.5in,BUTTONHEAD,BOLT:26 ↔ PLATE,HOOD,SIDE:2
- Mate:120: PLATE,SHOOTER,SIDE:1 ↔ PLATE,SHOOTER,BOTTOM:1
- Mate:121: PURCHASED,HEX_BEARING:14 ↔ STOCK,SHAFT,HEX,HOOD,WHEELS,LONG:1
- Mate:122: PURCHASED,HEX_BEARING:14 ↔ STOCK,SHAFT,HEX,HOOD,WHEELS,LONG:1
- Insert:94: PURCHASED,HEX_BEARING:15 ↔ PLATE,BEARING,MOUNT:1
- Insert:96: PURCHASED,HEX_BEARING:14 ↔ PLATE,BEARING,MOUNT:1
- Insert:98: PURCHASED,10-32x0.5in,BUTTONHEAD,BOLT:22 ↔ PLATE,BEARING,MOUNT:1
- Insert:99: PURCHASED,10-32x0.5in,BUTTONHEAD,BOLT:21 ↔ PLATE,BEARING,MOUNT:1
- Insert:100: PURCHASED,10-32x0.5in,BUTTONHEAD,BOLT:23 ↔ PLATE,BEARING,MOUNT:1
- Mate:124: PURCHASED,GEAR,20DP,30T,HEX:1 ↔ STOCK,SHAFT,HEX,HOOD,REVERSER:1
- Mate:125: PURCHASED,GEAR,20DP,30T,HEX:1 ↔ STOCK,SHAFT,HEX,HOOD,REVERSER:1
- Mate:126: PURCHASED,GEAR,20DP,30T,HEX:2 ↔ STOCK,SHAFT,HEX,HOOD,WHEELS,LONG:1
- Mate:127: PURCHASED,GEAR,20DP,30T,HEX:2 ↔ STOCK,SHAFT,HEX,HOOD,WHEELS,LONG:1
- Mate:128: PURCHASED,HEX_BEARING:7 ↔ PURCHASED,GEAR,20DP,30T,HEX:2
- Mate:129: PURCHASED,HEX_BEARING:12 ↔ PURCHASED,GEAR,20DP,30T,HEX:1
- Mate:131: 3DPRINT,BACKRAIL:1 ↔ PLATE,SHOOTER,BOTTOM:1
- Insert:101: PLATE,NUTBLOCK:1 ↔ PLATE,SHOOTER,SIDE:2
- Insert:102: PLATE,NUTBLOCK:1 ↔ PLATE,SHOOTER,BOTTOM:1
- Insert:103: PLATE,NUTBLOCK:2 ↔ PLATE,SHOOTER,BOTTOM:1
- Insert:104: PLATE,NUTBLOCK:2 ↔ PLATE,SHOOTER,SIDE:2
- Insert:107: PLATE,NUTBLOCK:4 ↔ PLATE,SHOOTER,BOTTOM:1
- Insert:110: PLATE,NUTBLOCK:5 ↔ PLATE,SHOOTER,SIDE:1
- Insert:111: PURCHASED,10-32x0.5in,BUTTONHEAD,BOLT:30 ↔ PLATE,SHOOTER,SIDE:1
- Insert:112: PURCHASED,10-32x0.5in,BUTTONHEAD,BOLT:29 ↔ PLATE,SHOOTER,SIDE:1
- Insert:113: PURCHASED,10-32x0.5in,BUTTONHEAD,BOLT:28 ↔ PLATE,SHOOTER,SIDE:1
- Insert:114: PURCHASED,10-32x0.5in,BUTTONHEAD,BOLT:27 ↔ PLATE,SHOOTER,SIDE:1
- Insert:115: PURCHASED,10-32x0.5in,BUTTONHEAD,BOLT:31 ↔ PLATE,SHOOTER,BOTTOM:1
- Insert:116: PURCHASED,10-32x0.5in,BUTTONHEAD,BOLT:32 ↔ PLATE,SHOOTER,BOTTOM:1
- Insert:117: PURCHASED,10-32x0.5in,BUTTONHEAD,BOLT:33 ↔ PLATE,SHOOTER,BOTTOM:1
- Insert:118: PURCHASED,10-32x0.5in,BUTTONHEAD,BOLT:34 ↔ PLATE,SHOOTER,BOTTOM:1
- Insert:119: PURCHASED,10-32x0.5in,BUTTONHEAD,BOLT:35 ↔ PLATE,SHOOTER,BOTTOM:1
- Insert:120: PURCHASED,10-32x0.5in,BUTTONHEAD,BOLT:36 ↔ PLATE,SHOOTER,BOTTOM:1
- Insert:121: PURCHASED,10-32x0.5in,BUTTONHEAD,BOLT:37 ↔ PLATE,SHOOTER,BOTTOM:1
- Insert:122: PURCHASED,10-32x0.5in,BUTTONHEAD,BOLT:38 ↔ PLATE,SHOOTER,BOTTOM:1
- Insert:124: PURCHASED,10-32x0.5in,BUTTONHEAD,BOLT:40 ↔ PLATE,SHOOTER,SIDE:2
- Insert:125: PURCHASED,10-32x0.5in,BUTTONHEAD,BOLT:41 ↔ PLATE,SHOOTER,SIDE:2
- Insert:126: PURCHASED,10-32x0.5in,BUTTONHEAD,BOLT:42 ↔ PLATE,SHOOTER,SIDE:2
- Insert:127: PURCHASED,10-32x0.5in,BUTTONHEAD,BOLT:43 ↔ PLATE,SHOOTER,SIDE:2
- Insert:128: PURCHASED,10-32x0.5in,BUTTONHEAD,BOLT:44 ↔ PLATE,SHOOTER,BACK:1
- Insert:129: PURCHASED,10-32x0.5in,BUTTONHEAD,BOLT:45 ↔ PLATE,SHOOTER,BACK:1
- Insert:137: PURCHASED,M4x12mm,BUTTONHEAD,BOLT:1 ↔ PLATE,SHOOTER,BOTTOM:1
- Insert:138: PURCHASED,M4x12mm,BUTTONHEAD,BOLT:2 ↔ PLATE,SHOOTER,BOTTOM:1
- Insert:139: PURCHASED,M4x12mm,BUTTONHEAD,BOLT:3 ↔ PLATE,SHOOTER,BOTTOM:1
- Insert:140: PURCHASED,M4x12mm,BUTTONHEAD,BOLT:4 ↔ PLATE,SHOOTER,BOTTOM:1
- Insert:141: PURCHASED,M4x12mm,BUTTONHEAD,BOLT:5 ↔ PLATE,SHOOTER,BOTTOM:1
- Insert:142: PURCHASED,M4x12mm,BUTTONHEAD,BOLT:6 ↔ PLATE,SHOOTER,BOTTOM:1
- Insert:143: PURCHASED,M4x12mm,BUTTONHEAD,BOLT:7 ↔ PLATE,SHOOTER,BOTTOM:1
- Insert:144: PURCHASED,M4x12mm,BUTTONHEAD,BOLT:8 ↔ PLATE,SHOOTER,BOTTOM:1
- Insert:145: PURCHASED,0.25-20x0.5in,BUTTONHEAD,BOLT:4 ↔ PLATE,SHOOTER,SIDE:2
- Insert:146: PURCHASED,0.25-20x0.5in,BUTTONHEAD,BOLT:1 ↔ PLATE,SHOOTER,SIDE:1
- Mate:141: PURCHASED,HTD5mm,20T,PULLEY:3 ↔ STOCK,SHAFT,HEX,SHOOTER:1
- Mate:142: PURCHASED,HTD5mm,20T,PULLEY:3 ↔ STOCK,SHAFT,HEX,SHOOTER:1
- Mate:144: PURCHASED,HTD5mm,20T,PULLEY:4 ↔ STOCK,SHAFT,HEX,HOOD,REVERSER:1
- Mate:145: PURCHASED,HTD5mm,20T,PULLEY:4 ↔ STOCK,SHAFT,HEX,HOOD,REVERSER:1
- Mate:146: PURCHASED,GEAR,20DP,30T,HEX:1 ↔ PURCHASED,HTD5mm,20T,PULLEY:4
- Mate:147: STANDIN,45T,HTD5mm,BELT:1 ↔ PLATE,HOOD,SIDE:2
- Mate:148: STANDIN,45T,HTD5mm,BELT:1 ↔ PLATE,HOOD,SIDE:2
- Mate:149: STANDIN,90T,HTD5mm,BELT:1 ↔ PLATE,SHOOTER,SIDE:2
- Mate:150: STANDIN,90T,HTD5mm,BELT:1 ↔ PLATE,HOOD,SIDE:2
- Mate:151 (0.75 mm): STANDIN,90T,HTD5mm,BELT:1 ↔ PURCHASED,HTD5mm,20T,PULLEY:4
- Mate:152 (0.75 mm): STANDIN,45T,HTD5mm,BELT:1 ↔ PURCHASED,HTD5mm,20T,PULLEY:1
- Flush:9: PURCHASED,HTD5mm,20T,PULLEY:3 ↔ STOCK,SHAFT,HEX,SHOOTER:1
- Mate:153: 3DPRINT,FLYWHEELTOHOOD,SPACER:1 ↔ STOCK,SHAFT,HEX,SHOOTER:1
- Mate:154: 3DPRINT,FLYWHEELTOHOOD,SPACER:1 ↔ STOCK,SHAFT,HEX,SHOOTER:1
- Mate:155: PURCHASED,HEX_BEARING:9 ↔ 3DPRINT,FLYWHEELTOHOOD,SPACER:1
- Insert:152: PLATE,HOOD,SIDE:1 ↔ STOCK,HOOD,SPACER,10-32,6.25in:1
- Insert:153: PLATE,HOOD,SIDE:2 ↔ STOCK,HOOD,SPACER,10-32,6.25in:2
- Insert:154: PURCHASED,10-32x0.5in,BUTTONHEAD,BOLT:49 ↔ PLATE,HOOD,SIDE:1
- Insert:155: PURCHASED,10-32x0.5in,BUTTONHEAD,BOLT:51 ↔ PLATE,HOOD,SIDE:1
- Insert:156: PURCHASED,10-32x0.5in,BUTTONHEAD,BOLT:50 ↔ PLATE,HOOD,SIDE:2
- Insert:157: PURCHASED,10-32x0.5in,BUTTONHEAD,BOLT:52 ↔ PLATE,HOOD,SIDE:2
- Mate:157: 3DPRINT,SIDEPLATETOHOOD,SPACER :1 ↔ STOCK,SHAFT,HEX,SHOOTER:1